# Autodesk Inventor assembly: structure_mirrored
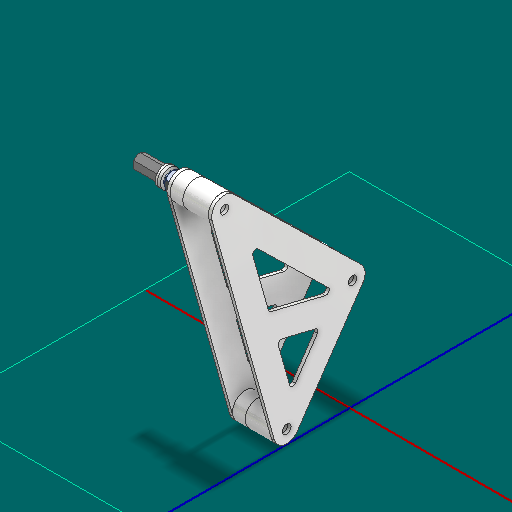
[picture p0: Inventor's stored thumbnail of the model, 512x512]
Saved by Autodesk Inventor 2025 (Build 290162000, 162)
## iProperties
Created: 2024-08-19
Part Number: structure_mirrored
Document SubType Name: Assembly
Designer: averey
Author: averey
## Documents named in this file (11)
- C:\Users\avere\vex_robotics_high_stakes\hardware\cad\ATLAS\tower\conveyer_box\structure_mirrored\structure_mirrored.iam
- C:\Users\avere\vex_robotics_high_stakes\hardware\cad\ATLAS\tower\conveyer_box\structure_mirrored\gusset_mirrored.ipt
- C:\Users\avere\vex_robotics_high_stakes\hardware\cad\VEX-CAD-Inventor\Motion\Spacers\Spacer Nylon .500 OD\NSpacer White .500 OD x .250.ipt
- C:\Users\avere\vex_robotics_high_stakes\hardware\cad\VEX-CAD-Inventor\Motion\Spacers\Spacer Nylon .500 OD.ipt
- C:\Users\avere\vex_robotics_high_stakes\hardware\cad\VEX-CAD-Inventor\Motion\Spacers\Spacer Nylon .500 OD\NSpacer White .500 OD x .500.ipt
- C:\Users\avere\vex_robotics_high_stakes\hardware\cad\ATLAS\tower\conveyer_box\structure_mirrored\Nut Thin Nylock_mirrored.ipt
- C:\Users\avere\vex_robotics_high_stakes\hardware\cad\VEX-CAD-Inventor\Motion\Spacers\Washer Teflon\TWasher .375 OD x .04000.ipt
- C:\Users\avere\vex_robotics_high_stakes\hardware\cad\VEX-CAD-Inventor\Motion\Spacers\Washer Teflon.ipt
- C:\Users\avere\vex_robotics_high_stakes\hardware\cad\VEX-CAD-Inventor\Structure\Standoff.ipt
- C:\Users\avere\vex_robotics_high_stakes\hardware\cad\VEX-CAD-Inventor\Structure\Standoff\Standoff .50.ipt
- C:\Users\avere\vex_robotics_high_stakes\hardware\cad\VEX-CAD-Inventor\Motion\Spacers\Washer Teflon\TWasher .375 OD x .06250.ipt
## Components (16 placed, 7 different names)
1. gusset_mirrored:1 — Insert:1, Mate:1, Insert:8, Insert:9
2. gusset_mirrored:2 — Insert:1, Mate:2, Mate:1, Insert:6, Insert:7, Insert:5
3. NSpacer White .500 OD x .250:1 — Insert:4
4. NSpacer White .500 OD x .500:2 — Insert:6, Insert:4
5. NSpacer White .500 OD x .250:3 — Insert:3
6. NSpacer White .500 OD x .500:4 — Insert:7, Insert:3
7. NSpacer White .500 OD x .250:5 — Insert:2
8. NSpacer White .500 OD x .500:6 — Insert:5, Insert:2
9. Nut Thin Nylock_mirrored:1 — Insert:8, Insert:24
10. Nut Thin Nylock_mirrored:2 — Insert:9, Insert:27
11. Standoff .50:3
12. TWasher .375 OD x .04000:3
13. TWasher .375 OD x .06250:4 — Insert:24
14. Standoff .50:4
15. TWasher .375 OD x .04000:5
16. TWasher .375 OD x .06250:6 — Insert:27
## Relationships (17: Insert 15, Mate 2)
- Insert:1 (19.05 mm): gusset_mirrored:1 ↔ gusset_mirrored:2
- Mate:2: gusset_mirrored:2
- Mate:1: gusset_mirrored:1 ↔ gusset_mirrored:2
- Insert:6: gusset_mirrored:2 ↔ NSpacer White .500 OD x .500:2
- Insert:4: NSpacer White .500 OD x .250:1 ↔ NSpacer White .500 OD x .500:2
- Insert:7: gusset_mirrored:2 ↔ NSpacer White .500 OD x .500:4
- Insert:3: NSpacer White .500 OD x .250:3 ↔ NSpacer White .500 OD x .500:4
- Insert:5: gusset_mirrored:2 ↔ NSpacer White .500 OD x .500:6
- Insert:2: NSpacer White .500 OD x .250:5 ↔ NSpacer White .500 OD x .500:6
- Insert:8: gusset_mirrored:1 ↔ Nut Thin Nylock_mirrored:1
- Insert:9: gusset_mirrored:1 ↔ Nut Thin Nylock_mirrored:2
- [Insert]: TWasher .375 OD x .04000:3 ↔ TWasher .375 OD x .06250:4
- [Insert]: Standoff .50:3 ↔ TWasher .375 OD x .04000:3
- Insert:24: Nut Thin Nylock_mirrored:1 ↔ TWasher .375 OD x .06250:4
- [Insert]: TWasher .375 OD x .04000:5 ↔ TWasher .375 OD x .06250:6
- [Insert]: Standoff .50:4 ↔ TWasher .375 OD x .04000:5
- Insert:27: Nut Thin Nylock_mirrored:2 ↔ TWasher .375 OD x .06250:6
## Named parameters: d26_d30 = 0 mm, d27_d31 = 0 mm
